# Autodesk Inventor assembly: ROV
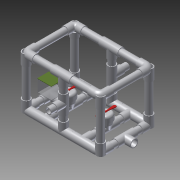
[picture p0: Inventor's stored thumbnail of the model, 180x180]
Saved by Autodesk Inventor 2013 (Build 170138000, 138)
## iProperties
Created: 2013-06-27
Part Number: ROV
Document SubType Name: Assembly
Designer: Kyle
Author: Kyle
## Documents named in this file (14)
- C:\Users\Kyle\Documents\Autodesk\Inventor\Projects\ROV\ROV.iam
- C:\Users\Kyle\Documents\Autodesk\Inventor\Projects\ROV\3 Way.ipt
- C:\Users\Kyle\Documents\Autodesk\Inventor\Projects\ROV\5in Pipe.ipt
- C:\Users\Kyle\Documents\Autodesk\Inventor\Projects\ROV\3in Pipe.ipt
- C:\Users\Kyle\Documents\Autodesk\Inventor\Projects\ROV\T.ipt
- C:\Users\Kyle\Documents\Autodesk\Inventor\Projects\ROV\2in Pipe.ipt
- C:\Users\Kyle\Documents\Autodesk\Inventor\Projects\ROV\T .75 to 1.ipt
- C:\Users\Kyle\Documents\Autodesk\Inventor\Projects\ROV\7in Pipe.ipt
- C:\Users\Kyle\Documents\Autodesk\Inventor\Projects\ROV\1.5in Pipe.ipt
- C:\Users\Kyle\Documents\Autodesk\Inventor\Projects\ROV\Cap.ipt
- C:\Users\Kyle\Documents\Autodesk\Inventor\Projects\ROV\Motor.ipt
- C:\Users\Kyle\Documents\Autodesk\Inventor\Projects\ROV\Prop.ipt
- C:\Users\Kyle\Documents\Autodesk\Inventor\Projects\ROV\Box.iam
- C:\Users\Kyle\Documents\Autodesk\Inventor\Projects\ROV\Motor End Cap.ipt
## Components (63 placed, 13 different names)
1. 3 Way:1 — Flush:1, Mate:7, Mate:8, Mate:16, Mate:18, Flush:4, Flush:5, Mate:125
2. 3 Way:2 — Flush:1, Mate:5, Mate:6, Mate:17, Mate:19, Flush:3, Angle:1, Flush:6, Mate:120, Mate:121, Angle:9
3. 5in Pipe:2 — Mate:5, Mate:6, Mate:9, Mate:10
4. 5in Pipe:3 — Mate:7, Mate:8, Mate:11, Mate:12
5. 3 Way:3 — Mate:9, Mate:10, Flush:2, Mate:13, Mate:39, Mate:41, Mate:119
6. 3 Way:4 — Mate:11, Flush:2, Mate:12, Mate:14, Mate:15, Mate:38, Mate:40
7. 5in Pipe:4 — Mate:13, Mate:14, Mate:15, Mate:119
8. 3in Pipe:1 — Mate:16, Mate:18, Mate:20, Mate:22
9. 3in Pipe:2 — Mate:17, Mate:19, Mate:21, Mate:23
10. T:1 — Mate:21, Mate:23, Flush:3, Mate:31, Mate:33, Flush:9
11. T:2 — Mate:20, Mate:22, Flush:4, Mate:24, Mate:25, Mate:30, Mate:32, Flush:8, Mate:148
12. 2in Pipe:1 — Mate:24, Mate:25, Mate:26
13. 2in Pipe:2 — Mate:28, Mate:29
14. T .75 to 1:1 — Mate:26, Mate:28, Mate:29, Angle:1, Flush:10, Mate:133, Flush:17, Mate:148
15. 3in Pipe:3 — Mate:30, Mate:32, Mate:34, Mate:36
16. 3in Pipe:5 — Mate:31, Mate:33, Mate:35, Mate:37
17. T:3 — Mate:34, Mate:36, Flush:5, Mate:42, Mate:43, Angle:2, Mate:70, Mate:72
18. T:4 — Mate:35, Mate:37, Flush:6, Mate:44, Mate:45, Angle:3, Mate:71, Mate:73
19. 7in Pipe:1 — Mate:38, Mate:40, Mate:54
20. 7in Pipe:2 — Mate:39, Mate:41, Mate:56
21. 2in Pipe:3 — Mate:42, Mate:43, Mate:46, Mate:48
22. 2in Pipe:4 — Mate:44, Mate:45, Mate:47, Mate:49
23. 2in Pipe:5 — Mate:50, Mate:51, Mate:55
24. 2in Pipe:6 — Mate:52, Mate:53, Mate:57
25. T:5 — Mate:46, Angle:2, Mate:48, Mate:50, Mate:51, Mate:58, Mate:59
26. T:6 — Mate:47, Angle:3, Mate:49, Mate:52, Mate:53, Mate:64, Mate:65
27. T:7 — Mate:54, Mate:55, Angle:7, Mate:105, Mate:106
28. T:8 — Mate:56, Mate:57, Angle:8, Mate:107, Mate:108
29. 1.5in Pipe:1 — Mate:58, Mate:59
30. 1.5in Pipe:2 — Mate:64, Mate:65
31. 3in Pipe:6 — Mate:71, Mate:73, Mate:75, Mate:77
32. 3in Pipe:7 — Mate:70, Mate:72, Mate:74, Mate:76
33. T:9 — Mate:74, Mate:76, Flush:8, Mate:78, Mate:79, Mate:84, Mate:86, Mate:149
34. T:10 — Mate:75, Mate:77, Flush:9, Mate:85, Mate:87
35. 2in Pipe:7 — Mate:78, Mate:79, Mate:80
36. 2in Pipe:8 — Mate:82, Mate:83
37. T .75 to 1:2 — Mate:80, Flush:10, Mate:82, Mate:83, Mate:132, Flush:16, Angle:11, Mate:149
38. 3in Pipe:8 — Mate:84, Mate:86, Mate:88, Mate:90
39. 3in Pipe:9 — Mate:85, Mate:87, Mate:89, Mate:91
40. 3 Way:5 — Mate:88, Flush:11, Mate:90, Mate:94, Mate:96, Mate:109, Mate:110
41. 3 Way:6 — Mate:89, Flush:11, Mate:91, Mate:95, Mate:97, Mate:113, Flush:12, Angle:12
42. 3 Way:7 — Mate:98, Mate:99, Angle:8
43. 3 Way:8 — Mate:100, Mate:101, Mate:102, Angle:7, Mate:103, Mate:104
44. 5in Pipe:6 — Mate:95, Mate:97, Mate:98, Mate:99
45. 5in Pipe:7 — Mate:94, Mate:96, Mate:100, Mate:101, Mate:102
46. 5in Pipe:8 — Mate:103, Mate:104
47. 7in Pipe:3 — Mate:105, Mate:106
48. 7in Pipe:4 — Mate:107, Mate:108
49. T:11 — Mate:111, Mate:112, Mate:114, Flush:12, Mate:115, Mate:116, Mate:118, Mate:138, Flush:22, Flush:23
50. 2in Pipe:9 — Mate:113, Mate:114
51. 2in Pipe:10 — Mate:109, Mate:110, Mate:111, Mate:112
52. 1.5in Pipe:3 — Mate:115, Mate:116, Mate:117
53. Cap:1 — Mate:117, Mate:118
54. T:12 — Mate:122, Mate:123, Mate:124, Mate:126, Angle:9
55. 2in Pipe:11 — Mate:120, Mate:121, Mate:122, Mate:123, Mate:124
56. 2in Pipe:12 — Mate:125, Mate:126
57. Motor:2 — Mate:132, Flush:16, Mate:136, Flush:20, Mate:144, Mate:145
58. Motor:4 — Mate:133, Flush:17, Mate:137, Flush:21, Mate:146, Mate:147
59. Prop:2 — Mate:136, Flush:20
60. Prop:4 — Mate:137, Flush:21
61. Box:1 [sub-assembly] — Mate:138, Angle:11, Angle:12, Flush:22, Flush:23
62. Motor End Cap:3 — Mate:144, Mate:145
63. Motor End Cap:4 — Mate:146, Mate:147
## Relationships (146: Mate 121, Flush 17, Angle 8)
- Flush:1: 3 Way:1 ↔ 3 Way:2
- Mate:5: 3 Way:2 ↔ 5in Pipe:2
- Mate:6 (-19.05 mm): 3 Way:2 ↔ 5in Pipe:2
- Mate:7: 3 Way:1 ↔ 5in Pipe:3
- Mate:8 (-19.05 mm): 3 Way:1 ↔ 5in Pipe:3
- Mate:9: 5in Pipe:2 ↔ 3 Way:3
- Mate:10 (-19.05 mm): 5in Pipe:2 ↔ 3 Way:3
- Mate:11: 5in Pipe:3 ↔ 3 Way:4
- Flush:2: 3 Way:3 ↔ 3 Way:4
- Mate:12 (-19.05 mm): 5in Pipe:3 ↔ 3 Way:4
- Mate:13: 3 Way:3 ↔ 5in Pipe:4
- Mate:14: 3 Way:4 ↔ 5in Pipe:4
- Mate:15 (-19.05 mm): 3 Way:4 ↔ 5in Pipe:4
- Mate:16: 3 Way:1 ↔ 3in Pipe:1
- Mate:17: 3 Way:2 ↔ 3in Pipe:2
- Mate:18 (-19.05 mm): 3 Way:1 ↔ 3in Pipe:1
- Mate:19 (-19.05 mm): 3 Way:2 ↔ 3in Pipe:2
- Mate:20: 3in Pipe:1 ↔ T:2
- Mate:21: 3in Pipe:2 ↔ T:1
- Mate:22 (-19.05 mm): 3in Pipe:1 ↔ T:2
- Mate:23 (-19.05 mm): 3in Pipe:2 ↔ T:1
- Flush:3: 3 Way:2 ↔ T:1
- Flush:4: 3 Way:1 ↔ T:2
- Mate:24: T:2 ↔ 2in Pipe:1
- Mate:25 (-19.05 mm): T:2 ↔ 2in Pipe:1
- Mate:26: 2in Pipe:1 ↔ T .75 to 1:1
- Mate:28: 2in Pipe:2 ↔ T .75 to 1:1
- Mate:29 (-19.05 mm): 2in Pipe:2 ↔ T .75 to 1:1
- Angle:1 (0 deg): 3 Way:2 ↔ T .75 to 1:1
- Mate:30: T:2 ↔ 3in Pipe:3
- Mate:31: T:1 ↔ 3in Pipe:5
- Mate:32 (-19.05 mm): T:2 ↔ 3in Pipe:3
- Mate:33 (-19.05 mm): T:1 ↔ 3in Pipe:5
- Mate:34: 3in Pipe:3 ↔ T:3
- Mate:35: 3in Pipe:5 ↔ T:4
- Mate:36 (-19.05 mm): 3in Pipe:3 ↔ T:3
- Mate:37 (-19.05 mm): 3in Pipe:5 ↔ T:4
- Flush:5: 3 Way:1 ↔ T:3
- Flush:6: 3 Way:2 ↔ T:4
- Mate:38: 3 Way:4 ↔ 7in Pipe:1
- Mate:39: 3 Way:3 ↔ 7in Pipe:2
- Mate:40 (-19.05 mm): 3 Way:4 ↔ 7in Pipe:1
- Mate:41 (-19.05 mm): 3 Way:3 ↔ 7in Pipe:2
- Mate:42: T:3 ↔ 2in Pipe:3
- Mate:43 (-19.05 mm): T:3 ↔ 2in Pipe:3
- Mate:44: T:4 ↔ 2in Pipe:4
- Mate:45 (-19.05 mm): T:4 ↔ 2in Pipe:4
- Mate:46: 2in Pipe:3 ↔ T:5
- Angle:2 (90 deg): T:3 ↔ T:5
- Mate:47: 2in Pipe:4 ↔ T:6
- Angle:3 (-90 deg): T:4 ↔ T:6
- Mate:48 (-19.05 mm): 2in Pipe:3 ↔ T:5
- Mate:49 (-19.05 mm): 2in Pipe:4 ↔ T:6
- Mate:50: 2in Pipe:5 ↔ T:5
- Mate:51 (-19.05 mm): 2in Pipe:5 ↔ T:5
- Mate:52: 2in Pipe:6 ↔ T:6
- Mate:53 (-19.05 mm): 2in Pipe:6 ↔ T:6
- Mate:54: 7in Pipe:1 ↔ T:7
- Mate:55: 2in Pipe:5 ↔ T:7
- Mate:56: 7in Pipe:2 ↔ T:8
- Mate:57: 2in Pipe:6 ↔ T:8
- Mate:58: T:5 ↔ 1.5in Pipe:1
- Mate:59 (-19.05 mm): T:5 ↔ 1.5in Pipe:1
- Mate:64: T:6 ↔ 1.5in Pipe:2
- Mate:65 (-19.05 mm): T:6 ↔ 1.5in Pipe:2
- Mate:70: T:3 ↔ 3in Pipe:7
- Mate:71: T:4 ↔ 3in Pipe:6
- Mate:72 (-19.05 mm): T:3 ↔ 3in Pipe:7
- Mate:73 (-19.05 mm): T:4 ↔ 3in Pipe:6
- Mate:74: 3in Pipe:7 ↔ T:9
- Mate:75: 3in Pipe:6 ↔ T:10
- Mate:76 (-19.05 mm): 3in Pipe:7 ↔ T:9
- Mate:77 (-19.05 mm): 3in Pipe:6 ↔ T:10
- Flush:8: T:2 ↔ T:9
- Flush:9: T:1 ↔ T:10
- Mate:78: T:9 ↔ 2in Pipe:7
- Mate:79 (-19.05 mm): T:9 ↔ 2in Pipe:7
- Mate:80: 2in Pipe:7 ↔ T .75 to 1:2
- Flush:10: T .75 to 1:1 ↔ T .75 to 1:2
- Mate:82: 2in Pipe:8 ↔ T .75 to 1:2
- Mate:83 (-19.05 mm): 2in Pipe:8 ↔ T .75 to 1:2
- Mate:84: T:9 ↔ 3in Pipe:8
- Mate:85: T:10 ↔ 3in Pipe:9
- Mate:86 (-19.05 mm): T:9 ↔ 3in Pipe:8
- Mate:87 (-19.05 mm): T:10 ↔ 3in Pipe:9
- Mate:88: 3in Pipe:8 ↔ 3 Way:5
- Mate:89: 3in Pipe:9 ↔ 3 Way:6
- Flush:11: 3 Way:5 ↔ 3 Way:6
- Mate:90 (-19.05 mm): 3in Pipe:8 ↔ 3 Way:5
- Mate:91 (-19.05 mm): 3in Pipe:9 ↔ 3 Way:6
- Mate:94: 3 Way:5 ↔ 5in Pipe:7
- Mate:95: 3 Way:6 ↔ 5in Pipe:6
- Mate:96 (-19.05 mm): 3 Way:5 ↔ 5in Pipe:7
- Mate:97 (-19.05 mm): 3 Way:6 ↔ 5in Pipe:6
- Mate:98: 3 Way:7 ↔ 5in Pipe:6
- Mate:99 (-19.05 mm): 3 Way:7 ↔ 5in Pipe:6
- Mate:100: 3 Way:8 ↔ 5in Pipe:7
- Mate:101: 3 Way:8 ↔ 5in Pipe:7
- Mate:102 (-19.05 mm): 3 Way:8 ↔ 5in Pipe:7
- Angle:7 (180 deg): T:7 ↔ 3 Way:8
- Angle:8 (0 deg): T:8 ↔ 3 Way:7
- Mate:103: 3 Way:8 ↔ 5in Pipe:8
- Mate:104 (-19.05 mm): 3 Way:8 ↔ 5in Pipe:8
- Mate:105: T:7 ↔ 7in Pipe:3
- Mate:106 (-19.05 mm): T:7 ↔ 7in Pipe:3
- Mate:107: T:8 ↔ 7in Pipe:4
- Mate:108 (-19.05 mm): T:8 ↔ 7in Pipe:4
- Mate:109: 3 Way:5 ↔ 2in Pipe:10
- Mate:110 (-19.05 mm): 3 Way:5 ↔ 2in Pipe:10
- Mate:111: T:11 ↔ 2in Pipe:10
- Mate:112 (-19.05 mm): T:11 ↔ 2in Pipe:10
- Mate:113: 3 Way:6 ↔ 2in Pipe:9
- Mate:114 (-19.05 mm): T:11 ↔ 2in Pipe:9
- Flush:12: 3 Way:6 ↔ T:11
- Mate:115: T:11 ↔ 1.5in Pipe:3
- Mate:116 (-19.05 mm): T:11 ↔ 1.5in Pipe:3
- Mate:117: 1.5in Pipe:3 ↔ Cap:1
- Mate:118: T:11 ↔ Cap:1
- Mate:119 (-19.05 mm): 3 Way:3 ↔ 5in Pipe:4
- Mate:120: 3 Way:2 ↔ 2in Pipe:11
- Mate:121 (-19.05 mm): 3 Way:2 ↔ 2in Pipe:11
- Mate:122: T:12 ↔ 2in Pipe:11
- Mate:123: T:12 ↔ 2in Pipe:11
- Mate:124 (-19.05 mm): T:12 ↔ 2in Pipe:11
- Mate:125: 3 Way:1 ↔ 2in Pipe:12
- Mate:126 (-19.05 mm): T:12 ↔ 2in Pipe:12
- Angle:9 (270 deg): 3 Way:2 ↔ T:12
- Mate:132: T .75 to 1:2 ↔ Motor:2
- Flush:16 (-6.35 mm): T .75 to 1:2 ↔ Motor:2
- Mate:133: T .75 to 1:1 ↔ Motor:4
- Flush:17 (-6.35 mm): T .75 to 1:1 ↔ Motor:4
- Mate:136: Motor:2 ↔ Prop:2
- Flush:20: Motor:2 ↔ Prop:2
- Mate:137: Motor:4 ↔ Prop:4
- Flush:21: Motor:4 ↔ Prop:4
- Mate:138: T:11 ↔ Box:1
- Angle:11 (0 deg): T .75 to 1:2 ↔ Box:1
- Angle:12 (0 deg): 3 Way:6 ↔ Box:1
- Flush:22 (-3.175 mm): T:11 ↔ Box:1
- Mate:144: Motor:2 ↔ Motor End Cap:3
- Mate:145: Motor:2 ↔ Motor End Cap:3
- Mate:146: Motor:4 ↔ Motor End Cap:4
- Mate:147: Motor:4 ↔ Motor End Cap:4
- Flush:23: T:11 ↔ Box:1
- Mate:148 (14.605 mm): T:2 ↔ T .75 to 1:1
- Mate:149 (14.605 mm): T:9 ↔ T .75 to 1:2
